# Autodesk Inventor assembly: TheLightWithinYou-Assembly
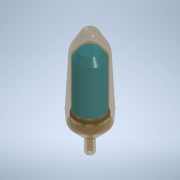
[picture p0: Inventor's stored thumbnail of the model, 180x180]
Saved by Autodesk Inventor 2021 (Build 250183000, 183)
## iProperties
Created: 2021-08-11
Part Number: TheLightWithinYou-Assembly
Document SubType Name: Assembly
Designer: incep
Author: incep
## Documents named in this file (5)
- C:\Users\incep\Desktop\3D Printer Stuff\TheLightWithinYou\TheLightWithinYou-Assembly.iam
- C:\Users\incep\Desktop\3D Printer Stuff\TheLightWithinYou\Bottom.ipt
- C:\Users\incep\Desktop\3D Printer Stuff\TheLightWithinYou\Flashbulb.ipt
- C:\Users\incep\Desktop\3D Printer Stuff\TheLightWithinYou\Upper.ipt
- C:\Users\incep\Desktop\3D Printer Stuff\TheLightWithinYou\R-22-O-ring.ipt
## Components (4 placed, 4 different names)
1. Bottom:1 — Mate:1, Mate:2, Mate:3, Mate:4, Mate:5, Mate:6
2. Flashbulb:1 — Mate:1, Mate:2, Mate:3
3. Upper:1 — Mate:4, Mate:5
4. R-22-O-ring:1 — Mate:6
## Relationships (6: Mate 6)
- Mate:1: Bottom:1 ↔ Flashbulb:1
- Mate:2: Bottom:1 ↔ Flashbulb:1
- Mate:3: Bottom:1 ↔ Flashbulb:1
- Mate:4: Bottom:1 ↔ Upper:1
- Mate:5: Bottom:1 ↔ Upper:1
- Mate:6: Bottom:1 ↔ R-22-O-ring:1
